# Autodesk Inventor assembly: Chassis
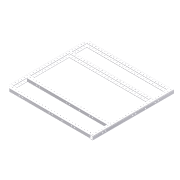
[picture p0: Inventor's stored thumbnail of the model, 180x180]
Saved by Autodesk Inventor 2014 SP1 (Build 180222100, 222)
## iProperties
Created: 2014-01-15
Part Number: Chassis
Document SubType Name: Assembly
Designer: Pradhan Alexander
Author: Pradhan Alexander
## Documents named in this file (4)
- K:\MHS\Technology\Holliday B\Group Projects\Robotics\CAD Team\CAD Team 2014\Chassis 2014\Chassis.iam
- K:\MHS\Technology\Holliday B\Group Projects\Robotics\CAD Team\CAD Team 2014\Chassis 2014\Chassis_Channel_AndyMark_am-0202-27in.ipt
- K:\MHS\Technology\Holliday B\Group Projects\Robotics\CAD Team\CAD Team 2014\Chassis 2014\Chassis_Channel_AndyMark_am-0202-27in-45.ipt
- K:\MHS\Technology\Holliday B\Group Projects\Robotics\CAD Team\CAD Team 2014\Chassis 2014\Chassis_Channel_AndyMark_am-0202-26.875.ipt
## Components (6 placed, 3 different names)
1. Chassis_Channel_AndyMark_am-0202-27in:2 — Mate:8, Flush:14, Flush:15, Flush:20, Flush:21
2. Chassis_Channel_AndyMark_am-0202-27in-45:1 — Mate:1, Flush:1, Flush:2, Mate:6, Flush:7, Mate:7, Flush:9, Mate:11, Angle:2, Mate:13, Angle:3, Mate:17, Flush:18, Flush:19
3. Chassis_Channel_AndyMark_am-0202-26.875:1 — Mate:7, Flush:9, Mate:9
4. Chassis_Channel_AndyMark_am-0202-26.875:2 — Mate:17, Flush:18, Flush:19, Flush:20, Flush:21
5. Chassis_Channel_AndyMark_am-0202-26.875:3 — Mate:1, Flush:1, Flush:2, Mate:8, Flush:14, Flush:15
6. Chassis_Channel_AndyMark_am-0202-26.875:4 — Mate:6, Flush:7, Mate:14, Angle:4
## Relationships (28: Mate 13, Flush 12, Angle 3)
- Mate:1: Chassis_Channel_AndyMark_am-0202-27in-45:1 ↔ Chassis_Channel_AndyMark_am-0202-26.875:3
- Flush:1: Chassis_Channel_AndyMark_am-0202-27in-45:1 ↔ Chassis_Channel_AndyMark_am-0202-26.875:3
- Flush:2: Chassis_Channel_AndyMark_am-0202-27in-45:1 ↔ Chassis_Channel_AndyMark_am-0202-26.875:3
- Mate:6: Chassis_Channel_AndyMark_am-0202-27in-45:1 ↔ Chassis_Channel_AndyMark_am-0202-26.875:4
- Flush:7: Chassis_Channel_AndyMark_am-0202-27in-45:1 ↔ Chassis_Channel_AndyMark_am-0202-26.875:4
- Mate:7: Chassis_Channel_AndyMark_am-0202-27in-45:1 ↔ Chassis_Channel_AndyMark_am-0202-26.875:1
- Flush:9: Chassis_Channel_AndyMark_am-0202-27in-45:1 ↔ Chassis_Channel_AndyMark_am-0202-26.875:1
- Mate:8: Chassis_Channel_AndyMark_am-0202-27in:2 ↔ Chassis_Channel_AndyMark_am-0202-26.875:3
- Flush:14: Chassis_Channel_AndyMark_am-0202-27in:2 ↔ Chassis_Channel_AndyMark_am-0202-26.875:3
- Flush:15: Chassis_Channel_AndyMark_am-0202-27in:2 ↔ Chassis_Channel_AndyMark_am-0202-26.875:3
- Mate:9: Chassis_Channel_AndyMark_am-0202-26.875:1
- Mate:10
- Mate:11: Chassis_Channel_AndyMark_am-0202-27in-45:1
- Mate:12
- Angle:2 (90 deg): Chassis_Channel_AndyMark_am-0202-27in-45:1
- Flush:16
- Mate:13: Chassis_Channel_AndyMark_am-0202-27in-45:1
- Mate:14: Chassis_Channel_AndyMark_am-0202-26.875:4
- Mate:15
- Angle:3 (90 deg): Chassis_Channel_AndyMark_am-0202-27in-45:1
- Mate:16
- Angle:4 (0 deg): Chassis_Channel_AndyMark_am-0202-26.875:4
- Flush:17
- Mate:17: Chassis_Channel_AndyMark_am-0202-27in-45:1 ↔ Chassis_Channel_AndyMark_am-0202-26.875:2
- Flush:18: Chassis_Channel_AndyMark_am-0202-27in-45:1 ↔ Chassis_Channel_AndyMark_am-0202-26.875:2
- Flush:19: Chassis_Channel_AndyMark_am-0202-27in-45:1 ↔ Chassis_Channel_AndyMark_am-0202-26.875:2
- Flush:20: Chassis_Channel_AndyMark_am-0202-27in:2 ↔ Chassis_Channel_AndyMark_am-0202-26.875:2
- Flush:21: Chassis_Channel_AndyMark_am-0202-27in:2 ↔ Chassis_Channel_AndyMark_am-0202-26.875:2
